# Autodesk Inventor assembly: Assembly Box
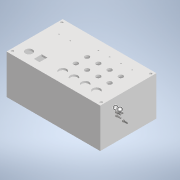
[picture p0: Inventor's stored thumbnail of the model, 180x180]
Saved by Autodesk Inventor 2022 (Build 260153000, 153)
## iProperties
Created: 2021-07-04
Part Number: Assembly Box
Document SubType Name: Assembly
Designer: Matthijs
Author: Matthijs
## Documents named in this file (4)
- C:\Users\Matthijs\Documents\Main_Files\DIY\ButtonBox 3D Parts\Assembly Box.iam
- C:\Users\Matthijs\Documents\Main_Files\DIY\ButtonBox 3D Parts\Box Top.ipt
- C:\Users\Matthijs\Documents\Main_Files\DIY\ButtonBox 3D Parts\Box.ipt
- C:\Users\Matthijs\Documents\Inventor\Content Center Files\R2022\en-US\ISO 4762(2)\ISO 4762 - M3 x 10ISO.ipt
## Components (6 placed, 3 different names)
1. Box Top:1 — Flush:1, Flush:2, Mate:1
2. Box:1 — Flush:1, Flush:2, Mate:1
3. ISO 4762 M3 x 10:1
4. ISO 4762 M3 x 10:2
5. ISO 4762 M3 x 10:3
6. ISO 4762 M3 x 10:4
## Relationships (3: Flush 2, Mate 1)
- Flush:1: Box Top:1 ↔ Box:1
- Flush:2: Box Top:1 ↔ Box:1
- Mate:1: Box Top:1 ↔ Box:1
